# Autodesk Inventor assembly: Assembly2
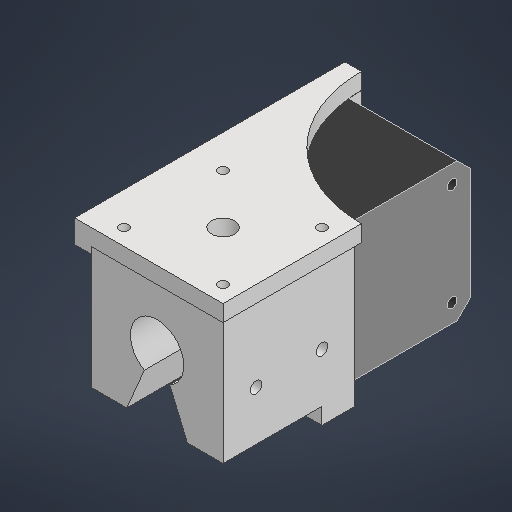
[picture p0: Inventor's stored thumbnail of the model, 512x512]
Saved by Autodesk Inventor 2025.1 (Build 291241000, 241)
## iProperties
Created: 2025-02-02
Part Number: Assembly2
Document SubType Name: Assembly
Designer: jerem
Author: jerem
## Documents named in this file (5)
- C:\Users\jerem\Documents\GitHub\Perovskite-Automated-Synthesis-System\CAD\Gantry\Assembly2 - Copy.iam
- C:\Users\jerem\Documents\GitHub\Perovskite-Automated-Synthesis-System\CAD\Gantry\X Axis End.ipt
- C:\Users\jerem\Documents\GitHub\Perovskite-Automated-Synthesis-System\CAD\Non 3D Printed Parts\Motors and Servos\NEMA17 Stepper Motor.ipt
- C:\Users\jerem\Documents\GitHub\Perovskite-Automated-Synthesis-System\CAD\Non 3D Printed Parts\Idler.ipt
- C:\Users\jerem\Documents\GitHub\Perovskite-Automated-Synthesis-System\CAD\Gantry\otherholderthing.ipt
## Components (4 placed, 4 different names)
1. X Axis End:1 — Mate:13, Mate:14, Flush:1, Mate:16
2. NEMA17 Stepper Motor:1 — Mate:5, Mate:14, Flush:1, Mate:15, Mate:17
3. Idler:1 — Mate:5, Mate:13
4. otherholderthing:1 — Mate:15, Mate:16, Mate:17
## Relationships (7: Mate 6, Flush 1)
- Mate:5: NEMA17 Stepper Motor:1 ↔ Idler:1
- Mate:13 (8 mm): X Axis End:1 ↔ Idler:1
- Mate:14: X Axis End:1 ↔ NEMA17 Stepper Motor:1
- Flush:1: X Axis End:1 ↔ NEMA17 Stepper Motor:1
- Mate:15: NEMA17 Stepper Motor:1 ↔ otherholderthing:1
- Mate:16: X Axis End:1 ↔ otherholderthing:1
- Mate:17: NEMA17 Stepper Motor:1 ↔ otherholderthing:1
